# Autodesk Inventor assembly: Giuntura
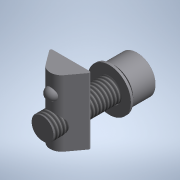
[picture p0: Inventor's stored thumbnail of the model, 180x180]
Saved by Autodesk Inventor 2022 (Build 260153000, 153)
## iProperties
Created: 2021-12-29
Part Number: Giuntura
Document SubType Name: Assembly
Designer: matte
Author: matte
## Documents named in this file (4)
- C:\Users\matte\Documents\GitHub\MDM-CyberOrto-CAD\Pezzi singoli\Supporto lineare\Giuntura.iam
- C:\Users\matte\Documents\GitHub\MDM-CyberOrto-CAD\Parker components\02-Fasteners\10-Standard T-Nuts\20-058.ipt
- C:\Users\matte\Documents\GitHub\MDM-CyberOrto-CAD\Parker components\02-Fasteners\15-T-Bolts_Nuts_Washers\03-Washers\24-708-8.ipt
- C:\Users\matte\Documents\GitHub\MDM-CyberOrto-CAD\Parker components\02-Fasteners\16-Screws\01-Metric Screws\03-Socket Head\24-325-8.ipt
## Components (3 placed, 3 different names)
1. 20-058:1 — Coincidente:4
2. 24-708-8:1 — Coincidente:4
3. 24-325-8:1
## Relationships (4: Mate 4)
- [Mate]: 20-058:1 ↔ 24-325-8:1
- [Mate]: 24-708-8:1 ↔ 24-325-8:1
- [Mate] (1 mm): 24-708-8:1 ↔ 24-325-8:1
- Coincidente:4 [Mate] (12 mm): 20-058:1 ↔ 24-708-8:1
